# Autodesk Inventor assembly: Assembly1
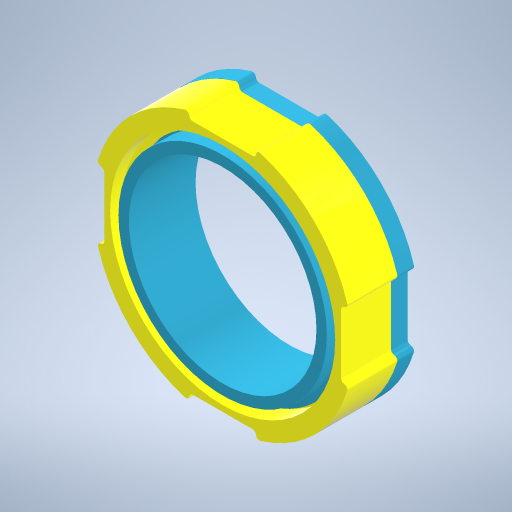
[picture p0: Inventor's stored thumbnail of the model, 512x512]
Saved by Autodesk Inventor 2023.2 (Build 272271030, 271C)
## iProperties
Created: 2023-10-23
Part Number: Assembly1
Document SubType Name: Assembly
Designer: Cris Pat
Author: Cris Pat
## Documents named in this file (3)
- C:\Users\Cris Pat\Desktop\U\Semestre_10\Disenio_y_manufactura\proyecto2\Assembly1.iam
- C:\Users\Cris Pat\Desktop\U\Semestre_10\Disenio_y_manufactura\proyecto2\rosca_1.ipt
- C:\Users\Cris Pat\Desktop\U\Semestre_10\Disenio_y_manufactura\proyecto2\rosca_2.ipt
## Components (2 placed, 2 different names)
1. rosca_1:1 — Rotational:1
2. rosca_2:1 — Rotational:1
## Relationships (1: RevoluteJoint 1)
- Rotational:1 [RevoluteJoint]: rosca_1:1 ↔ rosca_2:1
